# Autodesk Inventor assembly: Chassisv1
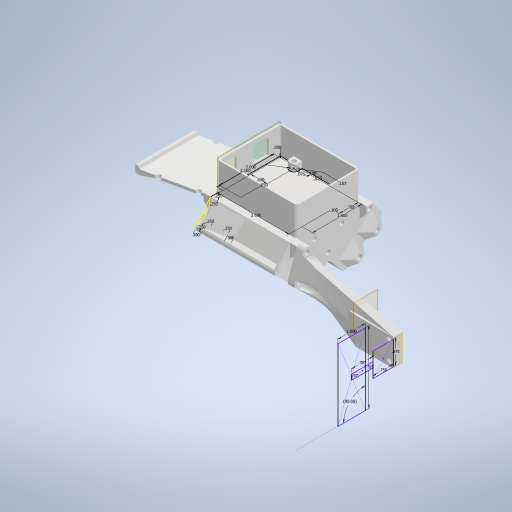
[picture p0: Inventor's stored thumbnail of the model, 512x512]
Saved by Autodesk Inventor 2023 (Build 270158030, 158C)
## iProperties
Created: 2024-03-25
Part Number: Chassisv1
Document SubType Name: Assembly
Designer: lvrectanus0
Author: lvrectanus0
## Documents named in this file (5)
- C:\Users\lvrectanus0\Documents\Github\SPARKLabs-ArduinoProjects\project\CAD\Autodesk\Chassisv1.iam
- C:\Users\lvrectanus0\Documents\Github\SPARKLabs-ArduinoProjects\project\CAD\Autodesk\ArduinoHolder-v2.ipt
- C:\Users\lvrectanus0\Documents\Github\SPARKLabs-ArduinoProjects\project\CAD\Autodesk\BatteryMount-v1.ipt
- C:\Users\lvrectanus0\Documents\Github\SPARKLabs-ArduinoProjects\project\CAD\Autodesk\BreadboardHolderv1.ipt
- C:\Users\lvrectanus0\Documents\Github\SPARKLabs-ArduinoProjects\project\CAD\Autodesk\Exports\MotorController-v1.ipt
## Components (4 placed, 4 different names)
1. ArduinoHolder-v2:1 — Flush:1, Flush:2
2. BatteryMount-v1:1 — Flush:1, Flush:2, Flush:3, Flush:4
3. BreadboardHolderv1:1 — Flush:3
4. MotorController-v1:1 — Flush:4
## Relationships (4: Flush 4)
- Flush:1: ArduinoHolder-v2:1 ↔ BatteryMount-v1:1
- Flush:2: ArduinoHolder-v2:1 ↔ BatteryMount-v1:1
- Flush:3: BatteryMount-v1:1 ↔ BreadboardHolderv1:1
- Flush:4: BatteryMount-v1:1 ↔ MotorController-v1:1
